# Autodesk Inventor assembly: Hinge
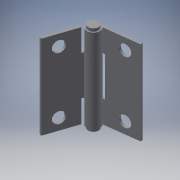
[picture p0: Inventor's stored thumbnail of the model, 180x180]
Saved by Autodesk Inventor 2016 (Build 200138000, 138)
## iProperties
Created: 2016-04-01
Part Number: Hinge
Document SubType Name: Assembly
Designer: amycroft3
Author: amycroft3
## Documents named in this file (4)
- C:\Users\Andrea\Documents\Dropbox\Capstone CAD\Hinge.iam
- C:\Users\Andrea\Documents\Dropbox\Capstone CAD\Hinge Pin.ipt
- C:\Users\Andrea\Documents\Dropbox\Capstone CAD\Hinge Wall 1.ipt
- C:\Users\Andrea\Documents\Dropbox\Capstone CAD\Hinge Wall 2.ipt
## Components (3 placed, 3 different names)
1. Hinge Pin:1 — Mate:1, Mate:2, Mate:3, Mate:4, Flush:2
2. Hinge Wall 1:1 — Mate:3, Flush:1, Flush:2
3. Hinge Wall 2:1 — Flush:1, Mate:4
## Relationships (6: Mate 4, Flush 2)
- Mate:1: Hinge Pin:1
- Mate:2: Hinge Pin:1
- Mate:3: Hinge Pin:1 ↔ Hinge Wall 1:1
- Flush:1: Hinge Wall 1:1 ↔ Hinge Wall 2:1
- Mate:4: Hinge Pin:1 ↔ Hinge Wall 2:1
- Flush:2 (-1.27 mm): Hinge Pin:1 ↔ Hinge Wall 1:1
